# Autodesk Inventor assembly: PT-100-775-CY-WH-LA
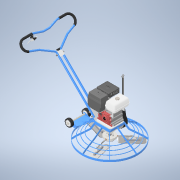
[picture p0: Inventor's stored thumbnail of the model, 180x180]
Saved by Autodesk Inventor 2021.1 (Build 251245010, 245A)
## iProperties
Company: Autodesk
RuleStatus: InUse
Created: 2020-08-27
Part Number: PT-100-775-CY-WH-LA
Document SubType Name: Assembly
Designer: alid
Catalog Web Link: www.autodesk.co.uk
Description: Power Trowel
Project: ADSK
Cost Center: 1066
Vendor: Autodesk
Engineer: alid
Stock Number: PWTR-0000
Author: alid
Title: Construction Tool
Revision Number: A
## Documents named in this file (27)
- C:\Users\peter\source\repos\InventorDA-FLC\Dataset\FY2021 Power Trowel\PWTR-0000.iam
- C:\Users\peter\source\repos\InventorDA-FLC\Dataset\FY2021 Power Trowel\PWTR-0001.ipt
- C:\Users\peter\source\repos\InventorDA-FLC\Dataset\FY2021 Power Trowel\PWTR-0023.iam
- C:\Users\peter\source\repos\InventorDA-FLC\Dataset\FY2021 Power Trowel\PWTR-0045.ipt
- C:\Users\peter\source\repos\InventorDA-FLC\Dataset\FY2021 Power Trowel\PWTR-0050.iam
- C:\Users\peter\source\repos\InventorDA-FLC\Dataset\FY2021 Power Trowel\PWTR-0062.ipt
- C:\Users\peter\source\repos\InventorDA-FLC\Dataset\FY2021 Power Trowel\PWTR-0063.ipt
- C:\Users\peter\source\repos\InventorDA-FLC\Dataset\FY2021 Power Trowel\PWTR-0064.ipt
- C:\Users\peter\source\repos\InventorDA-FLC\Dataset\FY2021 Power Trowel\PWTR-0066.ipt
- C:\Users\peter\source\repos\InventorDA-FLC\Dataset\FY2021 Power Trowel\PWTR-0067.ipt
- C:\Users\peter\source\repos\InventorDA-FLC\Dataset\FY2021 Power Trowel\PWTR-0068.ipt
- C:\Users\peter\source\repos\InventorDA-FLC\Dataset\FY2021 Power Trowel\PWTR-0069.ipt
- C:\Users\peter\source\repos\InventorDA-FLC\Dataset\FY2021 Power Trowel\PWTR-0070.ipt
- C:\Users\peter\source\repos\InventorDA-FLC\Dataset\FY2021 Power Trowel\PWTR-0071.ipt
- C:\Users\peter\source\repos\InventorDA-FLC\Dataset\FY2021 Power Trowel\PWTR-0072.ipt
- C:\Users\peter\source\repos\InventorDA-FLC\Dataset\FY2021 Power Trowel\PWTR-0073.ipt
- C:\Users\peter\source\repos\InventorDA-FLC\Dataset\FY2021 Power Trowel\PWTR-0083.ipt
- C:\Users\peter\source\repos\InventorDA-FLC\Dataset\FY2021 Power Trowel\PWTR-0124.ipt
- C:\Users\peter\source\repos\InventorDA-FLC\Dataset\FY2021 Power Trowel\PWTR-0131.ipt
- C:\Users\peter\source\repos\InventorDA-FLC\Dataset\FY2021 Power Trowel\PWTR-0132.ipt
- C:\Users\peter\source\repos\InventorDA-FLC\Dataset\FY2021 Power Trowel\PWTR-0136.iam
- C:\Users\peter\source\repos\InventorDA-FLC\Dataset\FY2021 Power Trowel\PWTR-0141.iam
- C:\Users\peter\source\repos\InventorDA-FLC\Dataset\FY2021 Power Trowel\GX 100.iam
- C:\Users\peter\source\repos\InventorDA-FLC\Dataset\FY2021 Power Trowel\PWTR-0127.iam
- C:\Users\peter\source\repos\InventorDA-FLC\Dataset\FY2021 Power Trowel\PWTR-0145.iam
- C:\Users\peter\source\repos\InventorDA-FLC\Dataset\FY2021 Power Trowel\PWTR-0058.ipt
- C:\Users\peter\source\repos\InventorDA-FLC\Dataset\FY2021 Power Trowel\PWTR-0059.ipt
## Components (42 placed, 26 different names)
1. Transfer Case — Rigid:1, Insert:9, Mate:2, Mate:4, Insert:10, Rigid:3, Rigid:4, Rigid:5, Mate:15, Mate:16, Mate:215, Mate:216, Coupling100
2. PWTR-0058:1 — Angle:2, Mate:2, Mate:217, Rotation:1
3. PWTR-0059:1 — Mate:5, Mate:215, Rotation:1
4. Trowel Guard — Rigid:1, Rigid:5, Mate:29, Flush:95, Mate:30, Lift01, Centre100, Drive100, Align100, Wheel01, Wheel02, Wheel03
5. Trowel Assembly [sub-assembly] — Insert:4, Angle:2, Insert:7
6. Trowel Transfer Bonnet [sub-assembly] — Insert:4, Insert:5, Rigid:4, Insert:13, Mate:217
7. ArmAssem [sub-assembly] — ArmFace, ArmHole, ArmCentre
8. ArmPlate — ArmFace, ArmHole, ArmCentre
9. PWTR-0062:1 — Insert:6
10. PWTR-0063:1 — Insert:5, Insert:6
11. PWTR-0064:1 — Insert:7
12. PWTR-0071:1
13. PWTR-0066:1 — Insert:9, Insert:11
14. PWTR-0067:1 — Mate:4, Mate:5, Mate:216
15. PWTR-0068:1 — Insert:10
16. PWTR-0069:1 — Insert:11
17. PWTR-0070:1 — Rigid:3, Insert:12
18. Adapter Plate — Insert:14, Mate:29, Flush:95, Mate:30, Mount100
19. Engine [sub-assembly] — Mount100, Centre100, Drive100, Lift02, Lift03
20. Drive Unit [sub-assembly] — Back100, Align100, Coupling100
21. Lifting Arm [sub-assembly] — Lift01, Lift02, Lift03
22. Wheel Assembly [sub-assembly] — Wheel01, Wheel02, Wheel03
23. PWTR-0072:1 — Insert:12
24. PWTR-0072:2
25. PWTR-0072:3
26. PWTR-0072:4
27. PWTR-0072:5
28. PWTR-0072:6
29. PWTR-0072:7
30. PWTR-0072:8
31. PWTR-0073:1 — Insert:13
32. PWTR-0073:2
33. PWTR-0073:3
34. PWTR-0073:4
35. PWTR-0124:1 — Mate:15, Mate:16
36. PWTR-0124:2
37. PWTR-0124:3
38. PWTR-0124:4
39. PWTR-0132:1 — Insert:14
40. PWTR-0132:2
41. PWTR-0132:3
42. PWTR-0132:4
## Component patterns: Drive Unit Fasteners (8 elements), Paddle Fasteners (4 elements), Arm Pattern (4 elements), Fastener Pattern (4 elements)
## Relationships (45: Mate 17, Insert 11, Flush 8, WeldJoint 6, Angle 2, RelateRotation 1)
- Rigid:1 [WeldJoint]: Transfer Case ↔ Trowel Guard
- [WeldJoint]: Transfer Case ↔ Trowel Transfer Bonnet
- Insert:4: Trowel Assembly ↔ Trowel Transfer Bonnet
- Angle:2 (72 deg): PWTR-0058:1 ↔ Trowel Assembly
- Insert:5: Trowel Transfer Bonnet ↔ PWTR-0063:1
- Insert:6: PWTR-0062:1 ↔ PWTR-0063:1
- Insert:7: Trowel Assembly ↔ PWTR-0064:1
- [Insert]: PWTR-0064:1 ↔ PWTR-0071:1
- Insert:9: Transfer Case ↔ PWTR-0066:1
- Mate:2: Transfer Case ↔ PWTR-0058:1
- Mate:4: Transfer Case ↔ PWTR-0067:1
- Mate:5: PWTR-0059:1 ↔ PWTR-0067:1
- Insert:10: Transfer Case ↔ PWTR-0068:1
- Insert:11: PWTR-0066:1 ↔ PWTR-0069:1
- Rigid:3 [WeldJoint]: Transfer Case ↔ PWTR-0070:1
- Insert:12: PWTR-0070:1 ↔ PWTR-0072:1
- Rigid:4 [WeldJoint]: Transfer Case ↔ Trowel Transfer Bonnet
- Rigid:5 [WeldJoint]: Transfer Case ↔ Trowel Guard
- Insert:13: Trowel Transfer Bonnet ↔ PWTR-0073:1
- [WeldJoint]: Transfer Case ↔ ArmPlate
- Mate:15: Transfer Case ↔ PWTR-0124:1
- Mate:16 (30 mm): Transfer Case ↔ PWTR-0124:1
- Insert:14: Adapter Plate ↔ PWTR-0132:1
- Mate:29: Trowel Guard ↔ Adapter Plate
- Flush:95 (-10 mm): Trowel Guard ↔ Adapter Plate
- Mate:30: Trowel Guard ↔ Adapter Plate
- Lift01 [Angle] (180 deg): Trowel Guard ↔ Lifting Arm
- Mate:215: Transfer Case ↔ PWTR-0059:1
- Mate:216: Transfer Case ↔ PWTR-0067:1
- Mate:217: PWTR-0058:1 ↔ Trowel Transfer Bonnet
- Rotation:1 [RelateRotation] (1.533 ul): PWTR-0058:1 ↔ PWTR-0059:1
- Mount100 [Flush]: Adapter Plate ↔ Engine
- Centre100 [Flush]: Trowel Guard ↔ Engine
- Drive100 [Flush]: Trowel Guard ↔ Engine
- Back100 [Flush]: Drive Unit
- Align100 [Flush]: Trowel Guard ↔ Drive Unit
- Coupling100 [Mate]: Transfer Case ↔ Drive Unit
- ArmFace [Mate]: ArmAssem ↔ ArmPlate
- ArmHole [Mate]: ArmAssem ↔ ArmPlate
- ArmCentre [Mate]: ArmAssem ↔ ArmPlate
- Lift02 [Mate]: Engine ↔ Lifting Arm
- Lift03 [Mate]: Engine ↔ Lifting Arm
- Wheel01 [Flush]: Trowel Guard ↔ Wheel Assembly
- Wheel02 [Mate]: Trowel Guard ↔ Wheel Assembly
- Wheel03 [Flush]: Trowel Guard ↔ Wheel Assembly
